# Autodesk Inventor assembly: set of axle holders
Saved by Autodesk Inventor 2015 (Build 190159000, 159)
## iProperties
Created: 2014-10-04
Part Number: set of axle holders
Document SubType Name: Assembly
Designer: jesse
Author: jesse
## Documents named in this file (2)
- C:\Users\jesse\Desktop\robot\set of axle holders.iam
- C:\Users\jesse\Desktop\robot\axle holder.ipt
## Components (3 placed, 1 different names)
1. axle holder:1
2. axle holder:2
3. axle holder:3
## Component patterns: (3 elements, first: axle holder:1)
